# Autodesk Inventor assembly: Gear Hub
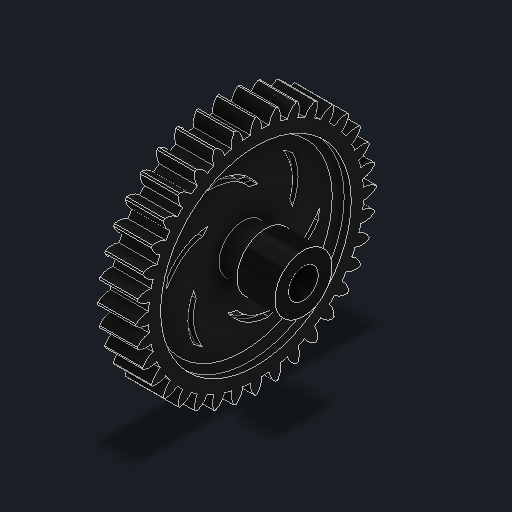
[picture p0: Inventor's stored thumbnail of the model, 512x512]
Saved by Autodesk Inventor 2025.1 (Build 291241000, 241)
## iProperties
Created: 2024-12-18
Part Number: Gear Hub
Document SubType Name: Assembly
Designer: avere
Author: avere
## Documents named in this file (4)
- C:\Users\avere\VEX\High Stakes\CAD\V4\Chassis\Drivebay Right\Gear Hub.iam
- C:\Users\avere\VEX\High Stakes\CAD\V4\Chassis\Drivebay Right\LS 36T Gear.ipt
- C:\Users\avere\VEX\High Stakes\CAD\ROBOPROS-CAD-Inventor\Motion\Spacers\Spacer Nylon .375 OD\NSpacer .375 OD x .250.ipt
- C:\Users\avere\VEX\High Stakes\CAD\ROBOPROS-CAD-Inventor\Motion\Spacers\Spacer Nylon .375 OD.ipt
## Components (2 placed, 2 different names)
1. LS 36T Gear:1 — Insert:1
2. NSpacer .375 OD x .250:1 — Insert:1
## Relationships (1: Insert 1)
- Insert:1: LS 36T Gear:1 ↔ NSpacer .375 OD x .250:1
